# Autodesk Inventor assembly: Ensamble EVA
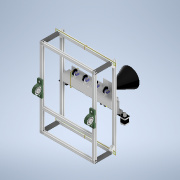
[picture p0: Inventor's stored thumbnail of the model, 180x180]
Saved by Autodesk Inventor 2022 (Build 260153000, 153)
## iProperties
Created: 2021-02-21
Part Number: Ensamble EVA
Document SubType Name: Assembly
Designer: juanp
Author: juanp
## Documents named in this file (9)
- C:\Users\juanp\OneDrive - Universidad de los andes\Uniandes\Robocol\EVA\V1  (Antiguo)\Ensamble EVA V1.iam
- C:\Users\juanp\OneDrive - Universidad de los andes\Uniandes\Robocol\EVA\Recursos\Actuador Lineal\Actuador Lineal (sin carro).iam
- C:\Users\juanp\OneDrive - Universidad de los andes\Uniandes\Robocol\EVA\Recursos\Chasis\Diseño 1.3 (2020)\Ensamble_chasis.iam
- C:\Users\juanp\OneDrive - Universidad de los andes\Uniandes\Robocol\EVA\Recursos\Actuador Lineal\Carro deslizante\Carro Deslizante.ipt
- C:\Users\juanp\OneDrive - Universidad de los andes\Uniandes\Robocol\EVA\V1  (Antiguo)\Dispensador\Dispensador V1.iam
- C:\Users\juanp\OneDrive - Universidad de los andes\Uniandes\Robocol\EVA\V1  (Antiguo)\Cajas\cajas.iam
- C:\Users\juanp\OneDrive - Universidad de los andes\Uniandes\Robocol\EVA\Recursos\Actuador Lineal\Partes\VSLOT 2020 Extrusion Mini.ipt
- C:\Users\juanp\OneDrive - Universidad de los andes\Uniandes\Robocol\EVA\Recursos\Pi Camera\RspCameraMia.iam
- C:\Users\juanp\OneDrive - Universidad de los andes\Uniandes\Robocol\EVA\V1  (Antiguo)\Camara\Case.ipt
## Components (9 placed, 8 different names)
1. Actuador Lineal (sin carro):1 [sub-assembly] — Angle:1, Angle:2, Mate:1, Angle:3, Angle:4, Flush:2, Mate:3, Flush:10, Mate:20, Mate:21, Mate:24
2. Ensamble_chasis:1 [sub-assembly] — Angle:1, Angle:2, Mate:1, Angle:5, Flush:11, Mate:19, Mate:23, Flush:13, Flush:15
3. Carro Deslizante:1 — Angle:3, Angle:4, Flush:2, Mate:3, Mate:4, Mate:5, Mate:6, Angle:6, Angle:7
4. Dispensador V1:1 [sub-assembly] — Mate:4, Mate:5, Mate:6, Mate:7, Mate:25, Mate:27, Mate:42, Mate:43
5. cajas:1 [sub-assembly] — Angle:5, Mate:7, Flush:10, Mate:25
6. VSLOT 2020 Extrusion Mini:1 — Flush:11, Mate:19, Mate:20, Mate:21, Flush:15
7. VSLOT 2020 Extrusion Mini:2 — Mate:23, Flush:13, Mate:24
8. RspCameraMia:1 [sub-assembly] — Angle:6, Mate:27, Mate:39, Mate:40, Mate:41
9. Case:1 — Mate:39, Mate:40, Mate:41, Angle:7, Mate:42, Mate:43
## Relationships (30: Mate 18, Angle 7, Flush 5)
- Angle:1 (180 deg): Actuador Lineal (sin carro):1 ↔ Ensamble_chasis:1
- Angle:2 (0 deg): Actuador Lineal (sin carro):1 ↔ Ensamble_chasis:1
- Mate:1: Actuador Lineal (sin carro):1 ↔ Ensamble_chasis:1
- Angle:3 (0 deg): Actuador Lineal (sin carro):1 ↔ Carro Deslizante:1
- Angle:4 (180 deg): Actuador Lineal (sin carro):1 ↔ Carro Deslizante:1
- Flush:2: Actuador Lineal (sin carro):1 ↔ Carro Deslizante:1
- Mate:3: Actuador Lineal (sin carro):1 ↔ Carro Deslizante:1
- Mate:4: Carro Deslizante:1 ↔ Dispensador V1:1
- Mate:5: Carro Deslizante:1 ↔ Dispensador V1:1
- Mate:6: Carro Deslizante:1 ↔ Dispensador V1:1
- Angle:5 (0 deg): Ensamble_chasis:1 ↔ cajas:1
- Mate:7 (4.167 mm): Dispensador V1:1 ↔ cajas:1
- Flush:10: Actuador Lineal (sin carro):1 ↔ cajas:1
- Flush:11: Ensamble_chasis:1 ↔ VSLOT 2020 Extrusion Mini:1
- Mate:19: Ensamble_chasis:1 ↔ VSLOT 2020 Extrusion Mini:1
- Mate:20: Actuador Lineal (sin carro):1 ↔ VSLOT 2020 Extrusion Mini:1
- Mate:21: Actuador Lineal (sin carro):1 ↔ VSLOT 2020 Extrusion Mini:1
- Mate:23: Ensamble_chasis:1 ↔ VSLOT 2020 Extrusion Mini:2
- Flush:13: Ensamble_chasis:1 ↔ VSLOT 2020 Extrusion Mini:2
- Mate:24: Actuador Lineal (sin carro):1 ↔ VSLOT 2020 Extrusion Mini:2
- Flush:15 (250 mm): Ensamble_chasis:1 ↔ VSLOT 2020 Extrusion Mini:1
- Mate:25: Dispensador V1:1 ↔ cajas:1
- Angle:6 (135 deg): Carro Deslizante:1 ↔ RspCameraMia:1
- Mate:27: Dispensador V1:1 ↔ RspCameraMia:1
- Mate:39: RspCameraMia:1 ↔ Case:1
- Mate:40: RspCameraMia:1 ↔ Case:1
- Mate:41: RspCameraMia:1 ↔ Case:1
- Angle:7 (0 deg): Carro Deslizante:1 ↔ Case:1
- Mate:42: Dispensador V1:1 ↔ Case:1
- Mate:43: Dispensador V1:1 ↔ Case:1
